# Autodesk Inventor assembly: Shoulder
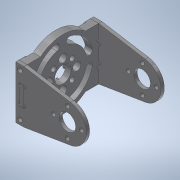
[picture p0: Inventor's stored thumbnail of the model, 180x180]
Saved by Autodesk Inventor 2020.4 (Build 244396000, 396)
## iProperties
Created: 2016-05-05
Part Number: Shoulder
Document SubType Name: Assembly
Designer: hiroaki
Mass: 31.2319 g
Surface Area: 187.261 cm^2
Volume: 14.2636 cm^3
Density: 2.18962 g/cm^3
Author: hiroaki
## Documents named in this file (3)
- C:\Users\Masato\Documents\Inventor\CIT Brains_Inventor\OpenPlatform_ver3_0\UpperBody\Arm\Shoulder.iam
- C:\Users\Masato\Documents\Inventor\CIT Brains_Inventor\OpenPlatform_ver3_0\UpperBody\Arm\Shoulder_vertical_frame_01.ipt
- C:\Users\Masato\Documents\Inventor\CIT Brains_Inventor\OpenPlatform_ver3_0\UpperBody\Arm\Shoulder_vertical_frame_02.ipt
## Components (3 placed, 2 different names)
1. Shoulder_vertical_frame_01:1 — 挿入:1, 挿入:2, 挿入:3, 挿入:4
2. Shoulder_vertical_frame_02:1 — 挿入:3, 挿入:4
3. Shoulder_vertical_frame_02:2 — 挿入:1, 挿入:2
## Relationships (4: Insert 4)
- 挿入:1 [Insert]: Shoulder_vertical_frame_01:1 ↔ Shoulder_vertical_frame_02:2
- 挿入:2 [Insert]: Shoulder_vertical_frame_01:1 ↔ Shoulder_vertical_frame_02:2
- 挿入:3 [Insert]: Shoulder_vertical_frame_01:1 ↔ Shoulder_vertical_frame_02:1
- 挿入:4 [Insert]: Shoulder_vertical_frame_01:1 ↔ Shoulder_vertical_frame_02:1
